# Autodesk Inventor assembly: washing_assembly
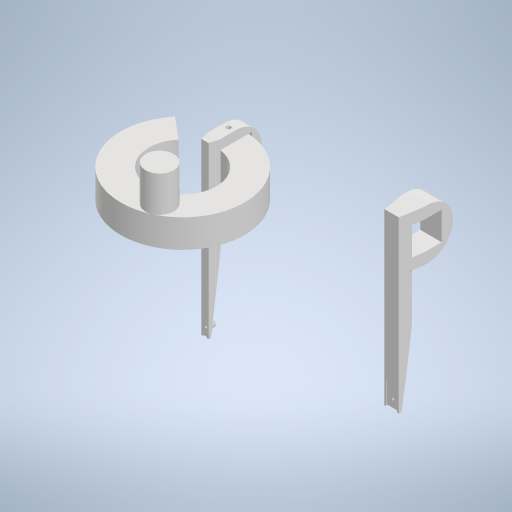
[picture p0: Inventor's stored thumbnail of the model, 512x512]
Saved by Autodesk Inventor 2023.4 (Build 274418000, 418)
## iProperties
Created: 2023-11-29
Part Number: washing_assembly
Document SubType Name: Assembly
Designer: mmelin
Author: mmelin
## Documents named in this file (4)
- X:\chronic_holder\washing\washing_assembly.iam
- X:\chronic_holder\washing\np2_washing_arm.ipt
- X:\chronic_holder\washing\wash_ring.ipt
- X:\chronic_holder\washing\np1_washing_arm.ipt
## Components (3 placed, 3 different names)
1. np2_washing_arm:1
2. wash_ring:1 — Flush:1
3. np1_washing_arm:2
## Relationships (1: Flush 1)
- Flush:1: wash_ring:1
